# Autodesk Inventor assembly: Podstawa_zlozona
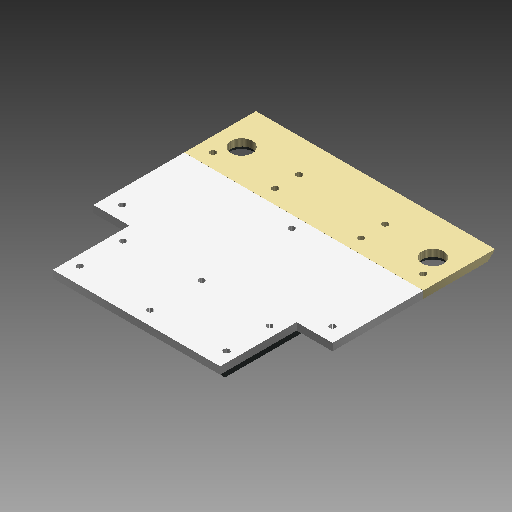
[picture p0: Inventor's stored thumbnail of the model, 512x512]
Saved by Autodesk Inventor 2017 (Build 210142000, 142)
## iProperties
Created: 2016-11-09
Part Number: Podstawa_zlozona
Document SubType Name: Assembly
Designer: Shichi
Author: Shichi
## Documents named in this file (4)
- C:\Users\Shichi\Desktop\TooStronk\Podstawy\Podstawa_zlozona.iam
- C:\Users\Shichi\Desktop\TooStronk\Podstawy\Podstawa.ipt
- C:\Users\Shichi\Desktop\TooStronk\Podstawy\Podstawa_Dolna.ipt
- C:\Users\Shichi\Desktop\TooStronk\Podstawy\Ostrze.ipt
## Components (3 placed, 3 different names)
1. Podstawa:1 — Insert:5, Insert:6, Insert:7, Insert:8
2. Podstawa_Dolna:1 — Insert:5, Insert:6
3. Ostrze:1 — Insert:7, Insert:8
## Relationships (4: Insert 4)
- Insert:5: Podstawa:1 ↔ Podstawa_Dolna:1
- Insert:6: Podstawa:1 ↔ Podstawa_Dolna:1
- Insert:7: Podstawa:1 ↔ Ostrze:1
- Insert:8: Podstawa:1 ↔ Ostrze:1
